# Autodesk Inventor assembly: AR-100
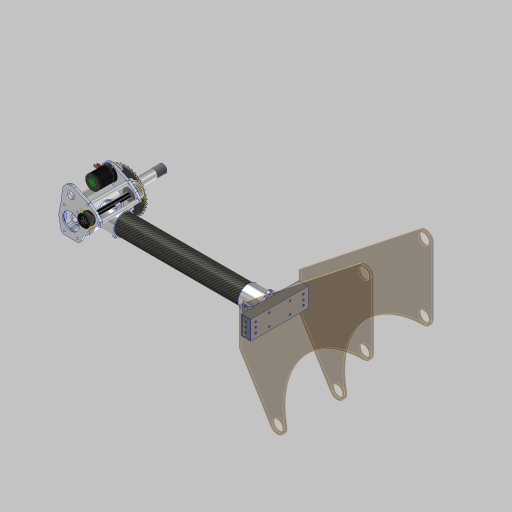
[picture p0: Inventor's stored thumbnail of the model, 512x512]
Saved by Autodesk Inventor 2023.5 (Build 275446000, 446)
## iProperties
Created: 2025-01-22
Part Number: AR-100
Document SubType Name: Assembly
Designer: slick
Mass: 2966.73 g
Surface Area: 9515.36 cm^2
Volume: 1838.81 cm^3
Density: 1.61339 g/cm^3
Author: slick
## Documents named in this file (20)
- C:\Users\slick\OneDrive\Desktop\2025-ReefScape---CAD\Arm\AR-100.iam
- C:\Users\slick\OneDrive\Desktop\2025-ReefScape---CAD\Arm\AR-001.ipt
- C:\Users\slick\OneDrive\Desktop\2025-ReefScape---CAD\Arm\AR-002.ipt
- C:\Users\slick\OneDrive\Desktop\2025-ReefScape---CAD\COMMON PARTS\BEARINGS\0_875_ID_x_1_875_OD_X_0_500_Radial_Bearing_EE11S-2RS.ipt
- C:\Users\slick\OneDrive\Desktop\2025-ReefScape---CAD\COMMON PARTS\MOTORS\Minion.ipt
- C:\Users\slick\OneDrive\Desktop\2025-ReefScape---CAD\COMMON PARTS\BEARINGS\13_75mm_1_2_ThunderHex_ID_x_1_125_OD_x_0_313_WD_Flanged_Bearing_217-4006_MIR.ipt
- C:\Users\slick\OneDrive\Desktop\2025-ReefScape---CAD\COMMON PARTS\PULLEYS\gt2\16T Gt2 Kracken PullyWCP-1178.ipt
- C:\Users\slick\OneDrive\Desktop\2025-ReefScape---CAD\COMMON PARTS\PULLEYS\gt2\36t_x_9mm_Wide_Double_Flange_Aluminum_Pulley_GT2_3mm_1_2_Hex_Bore_217-5873.ipt
- C:\Users\slick\OneDrive\Desktop\2025-ReefScape---CAD\Arm\AR-003.ipt
- C:\Users\slick\OneDrive\Desktop\2025-ReefScape---CAD\Arm\AR-005.ipt
- C:\Users\slick\OneDrive\Desktop\2025-ReefScape---CAD\Arm\AR-006.ipt
- C:\Users\slick\OneDrive\Desktop\2025-ReefScape---CAD\Arm\AR-007.ipt
- C:\Users\slick\OneDrive\Desktop\2025-ReefScape---CAD\COMMON PARTS\SPROCKETS\35\WCP-0983\WCP-0983.ipt
- C:\Users\slick\OneDrive\Desktop\2025-ReefScape---CAD\Arm\AR-009.ipt
- C:\Users\slick\OneDrive\Desktop\2025-ReefScape---CAD\Arm\AR-010.ipt
- C:\Users\slick\OneDrive\Desktop\2025-ReefScape---CAD\Gripper\GP3\GP3-100.iam
- C:\Users\slick\OneDrive\Desktop\2025-ReefScape---CAD\COMMON PARTS\PULLEYS\htd\18t_x_9mm_Wide_Double_Flange_Aluminum_Pulley_HTD_5mm_1_2_Hex_Bore_217-3225.ipt
- C:\Users\slick\OneDrive\Desktop\2025-ReefScape---CAD\Arm\AR-011.ipt
- C:\Users\slick\OneDrive\Desktop\2025-ReefScape---CAD\Arm\AR-012.ipt
- C:\Users\slick\OneDrive\Desktop\2025-ReefScape---CAD\Gripper\GP4\GP4-100.iam
## Components (22 placed, 19 different names)
1. AR-001:1 — Mate:1, Mate:2, Mate:3, Mate:4, Insert:1, Insert:2, Mate:13, Mate:14, Insert:29, Insert:30
2. AR-002:1 — Insert:1, Insert:2, Mate:5, Insert:4, Mate:8, Insert:5, Insert:19, Insert:20, Insert:28, Insert:33
3. 0_875_ID_x_1_875_OD_X_0_500_Radial_Bearing_EE11S-2RS:1 — Mate:1, Mate:3, Mate:15, Flush:2
4. 0_875_ID_x_1_875_OD_X_0_500_Radial_Bearing_EE11S-2RS:2 — Mate:2, Mate:4
5. Minion:1 — Mate:5, Mate:7, Flush:1, Mate:8, Insert:5
6. 13_75mm_1_2_ThunderHex_ID_x_1_125_OD_x_0_313_WD_Flanged_Bearing_217-4006_MIR:1 — Insert:4, Mate:9
7. 16T Gt2 Kracken PullyWCP-1178:1 — Mate:7, Flush:1, Mate:10
8. 36t_x_9mm_Wide_Double_Flange_Aluminum_Pulley_GT2_3mm_1_2_Hex_Bore_217-5873:1 — Mate:9, Mate:10
9. 13_75mm_1_2_ThunderHex_ID_x_1_125_OD_x_0_313_WD_Flanged_Bearing_217-4006_MIR:2 — Insert:14, Mate:19
10. AR-005:1 — Mate:13, Mate:14, Mate:17, Mate:18
11. AR-006:1 — Mate:15, Flush:2
12. AR-007:1 — Insert:14, Insert:31, Insert:32
13. AR-003:1 — Insert:28, Insert:31
14. AR-003:2 — Insert:32, Insert:33
15. WCP-0983:1 — Insert:21, Insert:22, Insert:23, Insert:24
16. AR-009:1 — Insert:19, Insert:20, Insert:21, Insert:22, Insert:23, Insert:24
17. AR-010:1 — Mate:17, Mate:18, Insert:25, Insert:26, Insert:34, Insert:35
18. GP3-100:1 [sub-assembly] — Insert:25, Insert:26, Flush:4
19. 18t_x_9mm_Wide_Double_Flange_Aluminum_Pulley_HTD_5mm_1_2_Hex_Bore_217-3225:1 — Mate:19, Flush:4, Mate:20, Flush:5
20. AR-011:1 — Insert:29, Insert:30
21. AR-012:1 — Mate:20, Flush:5
22. GP4-100:1 [sub-assembly] — Insert:34, Insert:35
## Relationships (41: Insert 21, Mate 16, Flush 4)
- Mate:1: AR-001:1 ↔ 0_875_ID_x_1_875_OD_X_0_500_Radial_Bearing_EE11S-2RS:1
- Mate:2: AR-001:1 ↔ 0_875_ID_x_1_875_OD_X_0_500_Radial_Bearing_EE11S-2RS:2
- Mate:3: AR-001:1 ↔ 0_875_ID_x_1_875_OD_X_0_500_Radial_Bearing_EE11S-2RS:1
- Mate:4: AR-001:1 ↔ 0_875_ID_x_1_875_OD_X_0_500_Radial_Bearing_EE11S-2RS:2
- Insert:1: AR-001:1 ↔ AR-002:1
- Insert:2: AR-001:1 ↔ AR-002:1
- Mate:5: AR-002:1 ↔ Minion:1
- Insert:4: AR-002:1 ↔ 13_75mm_1_2_ThunderHex_ID_x_1_125_OD_x_0_313_WD_Flanged_Bearing_217-4006_MIR:1
- Mate:7: Minion:1 ↔ 16T Gt2 Kracken PullyWCP-1178:1
- Flush:1: Minion:1 ↔ 16T Gt2 Kracken PullyWCP-1178:1
- Mate:8: AR-002:1 ↔ Minion:1
- Insert:5: AR-002:1 ↔ Minion:1
- Mate:9: 13_75mm_1_2_ThunderHex_ID_x_1_125_OD_x_0_313_WD_Flanged_Bearing_217-4006_MIR:1 ↔ 36t_x_9mm_Wide_Double_Flange_Aluminum_Pulley_GT2_3mm_1_2_Hex_Bore_217-5873:1
- Mate:10: 16T Gt2 Kracken PullyWCP-1178:1 ↔ 36t_x_9mm_Wide_Double_Flange_Aluminum_Pulley_GT2_3mm_1_2_Hex_Bore_217-5873:1
- Mate:13: AR-001:1 ↔ AR-005:1
- Mate:14 (-50.8 mm): AR-001:1 ↔ AR-005:1
- Mate:15: 0_875_ID_x_1_875_OD_X_0_500_Radial_Bearing_EE11S-2RS:1 ↔ AR-006:1
- Flush:2 (-12.7 mm): 0_875_ID_x_1_875_OD_X_0_500_Radial_Bearing_EE11S-2RS:1 ↔ AR-006:1
- Insert:14: 13_75mm_1_2_ThunderHex_ID_x_1_125_OD_x_0_313_WD_Flanged_Bearing_217-4006_MIR:2 ↔ AR-007:1
- Insert:19: AR-002:1 ↔ AR-009:1
- Insert:20: AR-002:1 ↔ AR-009:1
- Insert:21: WCP-0983:1 ↔ AR-009:1
- Insert:22: WCP-0983:1 ↔ AR-009:1
- Insert:23: WCP-0983:1 ↔ AR-009:1
- Insert:24: WCP-0983:1 ↔ AR-009:1
- Mate:17: AR-005:1 ↔ AR-010:1
- Mate:18: AR-005:1 ↔ AR-010:1
- Insert:25: AR-010:1 ↔ GP3-100:1
- Insert:26: AR-010:1 ↔ GP3-100:1
- Insert:28: AR-002:1 ↔ AR-003:1
- Mate:19: 13_75mm_1_2_ThunderHex_ID_x_1_125_OD_x_0_313_WD_Flanged_Bearing_217-4006_MIR:2 ↔ 18t_x_9mm_Wide_Double_Flange_Aluminum_Pulley_HTD_5mm_1_2_Hex_Bore_217-3225:1
- Flush:4: GP3-100:1 ↔ 18t_x_9mm_Wide_Double_Flange_Aluminum_Pulley_HTD_5mm_1_2_Hex_Bore_217-3225:1
- Insert:29: AR-001:1 ↔ AR-011:1
- Insert:30: AR-001:1 ↔ AR-011:1
- Mate:20: 18t_x_9mm_Wide_Double_Flange_Aluminum_Pulley_HTD_5mm_1_2_Hex_Bore_217-3225:1 ↔ AR-012:1
- Flush:5: 18t_x_9mm_Wide_Double_Flange_Aluminum_Pulley_HTD_5mm_1_2_Hex_Bore_217-3225:1 ↔ AR-012:1
- Insert:31: AR-007:1 ↔ AR-003:1
- Insert:32: AR-007:1 ↔ AR-003:2
- Insert:33: AR-002:1 ↔ AR-003:2
- Insert:34: AR-010:1 ↔ GP4-100:1
- Insert:35: AR-010:1 ↔ GP4-100:1
